# Autodesk Inventor assembly: TCSM1-220
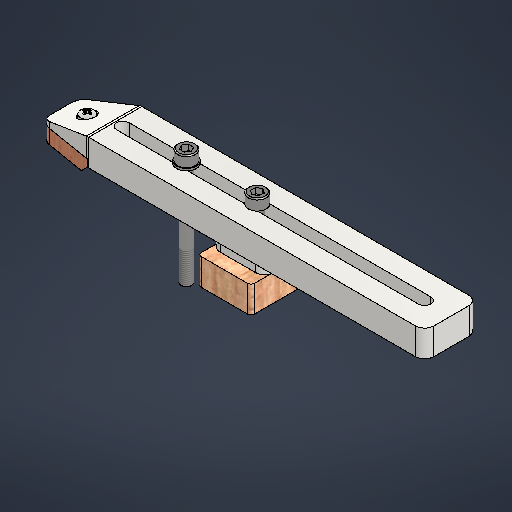
[picture p0: Inventor's stored thumbnail of the model, 512x512]
Saved by Autodesk Inventor 2025.3 (Build 293356000, 356)
## iProperties
Created: 2025-08-24
Part Number: TCSM1-220
Document SubType Name: Assembly
Designer: fablabadmin
Author: fablabadmin
## Documents named in this file (12)
- C:\Users\fablabadmin\Documents\_Benjamin_S\_3dCAD\HHVerkstad\ToeClampSM1\TCSM1-220.iam
- C:\Users\fablabadmin\Documents\_Benjamin_S\_3dCAD\HHVerkstad\ToeClampSM1\TCSM1-220-001.ipt
- C:\Users\fablabadmin\Documents\Inventor\Content Center Files\R2024\en-US\en-US\AS 1420\AS 1420 - 1973 - M4 x 8.ipt
- C:\Users\fablabadmin\Documents\Inventor\Content Center Files\R2024\en-US\en-US\AS 1420\AS 1420 - 1973 - M6 x 60.ipt
- C:\Users\fablabadmin\Documents\Inventor\Content Center Files\R2024\en-US\en-US\AS 1237 (2.1)\AS 1237 - 6.ipt
- C:\Users\fablabadmin\Documents\_Benjamin_S\_3dCAD\HHVerkstad\ToeClampSM1\TCSM1-X-003.ipt
- C:\Users\fablabadmin\Documents\_Benjamin_S\_3dCAD\HHVerkstad\ToeClampSM1\TCSM1-002B.ipt
- C:\Users\fablabadmin\Documents\_Benjamin_S\_3dCAD\HHVerkstad\ToeClampSM1\TCSM1-004.ipt
- C:\Users\fablabadmin\Documents\Inventor\Content Center Files\R2024\en-US\en-US\AS 1420\AS 1420 - 1973 - M6 x 16.ipt
- C:\Users\fablabadmin\Documents\_Benjamin_S\_3dCAD\HHVerkstad\ToeClampSM1\TCSM1-15-005.ipt
- C:\Users\fablabadmin\Documents\Inventor\Content Center Files\R2024\en-US\en-US\AS 1427(04)\AS 1427 - M4 x 10(5) I.ipt
- C:\Users\fablabadmin\Documents\Inventor\Content Center Files\R2024\en-US\en-US\DIN 7985 (H)\DIN 7985 (H) - M4x12-H.ipt
## Components (12 placed, 11 different names)
1. TCSM1-220-001:1 — Insert:1, Mate:7, Mate:11, Mate:12, Mate:13, Mate:14, Mate:16, Angle:1, Mate:22, Mate:23
2. AS 1420 - Metric M4 x 8:1 — Insert:1
3. AS 1420 - Metric M6 x 16:1 — Mate:7, Mate:15
4. AS 1420 - Metric M6 x 60:1 — Mate:8, Mate:9, Mate:10
5. AS 1237 (2.1) 6:1 — Mate:9, Mate:10, Mate:11
6. TCSM1-X-003:1
7. TCSM1-002B:1 — Mate:12, Mate:13, Mate:14
8. TCSM1-004:1 — Mate:15, Mate:16, Mate:17, Angle:1, Flush:2, Mate:18, Mate:20, Mate:21
9. TCSM1-15-005:1 — Flush:1, Flush:2, Mate:18
10. AS 1427 H - Metric M4 x 10:2 — Mate:20
11. AS 1427 H - Metric M4 x 10:1 — Mate:21
12. DIN 7985 (H) M4x12-H:1 — Mate:22, Mate:23
## Relationships (20: Mate 16, Flush 2, Insert 1, Angle 1)
- Insert:1: TCSM1-220-001:1 ↔ AS 1420 - Metric M4 x 8:1
- Mate:7: TCSM1-220-001:1 ↔ AS 1420 - Metric M6 x 16:1
- Mate:8: AS 1420 - Metric M6 x 60:1
- Mate:9: AS 1420 - Metric M6 x 60:1 ↔ AS 1237 (2.1) 6:1
- Mate:10: AS 1420 - Metric M6 x 60:1 ↔ AS 1237 (2.1) 6:1
- Mate:11: TCSM1-220-001:1 ↔ AS 1237 (2.1) 6:1
- Mate:12: TCSM1-220-001:1 ↔ TCSM1-002B:1
- Mate:13: TCSM1-220-001:1 ↔ TCSM1-002B:1
- Mate:14: TCSM1-220-001:1 ↔ TCSM1-002B:1
- Mate:15: AS 1420 - Metric M6 x 16:1 ↔ TCSM1-004:1
- Mate:16: TCSM1-220-001:1 ↔ TCSM1-004:1
- Mate:17: TCSM1-004:1
- Angle:1 (0 deg): TCSM1-220-001:1 ↔ TCSM1-004:1
- Flush:1: TCSM1-15-005:1
- Flush:2: TCSM1-004:1 ↔ TCSM1-15-005:1
- Mate:18: TCSM1-004:1 ↔ TCSM1-15-005:1
- Mate:20: TCSM1-004:1 ↔ AS 1427 H - Metric M4 x 10:2
- Mate:21: TCSM1-004:1 ↔ AS 1427 H - Metric M4 x 10:1
- Mate:22: TCSM1-220-001:1 ↔ DIN 7985 (H) M4x12-H:1
- Mate:23: TCSM1-220-001:1 ↔ DIN 7985 (H) M4x12-H:1
